# Autodesk Inventor assembly: 000.400 - Рычаг 2
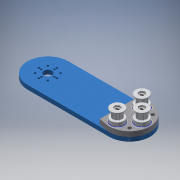
[picture p0: Inventor's stored thumbnail of the model, 180x180]
Saved by Autodesk Inventor 2019 (Build 230136000, 136)
## iProperties
Created: 2020-03-18
Part Number: 000.400 - Рычаг 2
Material: Типовые
Document SubType Name: Assembly
Designer: Петров Иван
Author: Петров Иван
## Documents named in this file (6)
- E:\IVAN\Ivan_desktop\GitHub\Manipulation_IRS\hardware\SCARA\000.400 - Рычаг 2.iam
- E:\IVAN\Ivan_desktop\GitHub\Manipulation_IRS\hardware\SCARA\000.401 - Опорная платформа.ipt
- E:\IVAN\Ivan_desktop\GitHub\Manipulation_IRS\hardware\SCARA\components\Подшипник 626Z.ipt
- E:\IVAN\Ivan_desktop\GitHub\Manipulation_IRS\hardware\SCARA\000.403 -  Прижим подшипников.ipt
- E:\IVAN\Ivan_desktop\GitHub\Manipulation_IRS\hardware\SCARA\components\Timing Pulley 18T.ipt
- C:\Users\Петров Иван\Documents\Inventor\Content Center Files\R2019\ru-RU\CNS 3129\CNS 3129 - M 4 x 0,7.ipt
## Components (11 placed, 5 different names)
1. 000.401 - Опорная платформа:1 — Совмещение:1, Совмещение:2, Совмещение:3, Совмещение:4, Совмещение:5, Совмещение:6, Совмещение:7
2. Подшипник 626Z:1 — Совмещение:1, Совмещение:6, Совмещение:8, Совмещение:14, Совмещение:15
3. Подшипник 626Z:2 — Совмещение:2, Совмещение:4, Совмещение:9, Совмещение:12, Совмещение:13
4. Подшипник 626Z:3 — Совмещение:3, Совмещение:5, Совмещение:10, Совмещение:11
5. 000.403 -  Прижим подшипников:1 — Совмещение:7, Совмещение:8, Совмещение:9
6. Timing Pulley 18T:1 — Совмещение:10, Совмещение:11, Направление навивки:2, Совмещение:18, Совмещение:19, Угол:3
7. Timing Pulley 18T:2 — Совмещение:14, Совмещение:15, Направление навивки:1, Совмещение:16, Угол:2, Совмещение:17
8. Timing Pulley 18T:3 — Совмещение:12, Совмещение:13, Направление навивки:1, Направление навивки:2, Вставка:1, Угол:1
9. CNS 3129 M 4:1 — Вставка:1, Угол:1
10. CNS 3129 M 4:2 — Совмещение:16, Угол:2, Совмещение:17
11. CNS 3129 M 4:3 — Совмещение:18, Совмещение:19, Угол:3
## Relationships (25: Mate 19, Angle 3, RelateRotation 2, Insert 1)
- Совмещение:1 [Mate]: 000.401 - Опорная платформа:1 ↔ Подшипник 626Z:1
- Совмещение:2 [Mate]: 000.401 - Опорная платформа:1 ↔ Подшипник 626Z:2
- Совмещение:3 [Mate]: 000.401 - Опорная платформа:1 ↔ Подшипник 626Z:3
- Совмещение:4 [Mate]: 000.401 - Опорная платформа:1 ↔ Подшипник 626Z:2
- Совмещение:5 [Mate]: 000.401 - Опорная платформа:1 ↔ Подшипник 626Z:3
- Совмещение:6 [Mate]: 000.401 - Опорная платформа:1 ↔ Подшипник 626Z:1
- Совмещение:7 [Mate]: 000.401 - Опорная платформа:1 ↔ 000.403 -  Прижим подшипников:1
- Совмещение:8 [Mate]: Подшипник 626Z:1 ↔ 000.403 -  Прижим подшипников:1
- Совмещение:9 [Mate]: Подшипник 626Z:2 ↔ 000.403 -  Прижим подшипников:1
- Совмещение:10 [Mate]: Подшипник 626Z:3 ↔ Timing Pulley 18T:1
- Совмещение:11 [Mate]: Подшипник 626Z:3 ↔ Timing Pulley 18T:1
- Совмещение:12 [Mate]: Подшипник 626Z:2 ↔ Timing Pulley 18T:3
- Совмещение:13 [Mate]: Подшипник 626Z:2 ↔ Timing Pulley 18T:3
- Совмещение:14 [Mate]: Подшипник 626Z:1 ↔ Timing Pulley 18T:2
- Совмещение:15 [Mate]: Подшипник 626Z:1 ↔ Timing Pulley 18T:2
- Направление навивки:1 [RelateRotation] (1 ul): Timing Pulley 18T:2 ↔ Timing Pulley 18T:3
- Направление навивки:2 [RelateRotation] (1 ul): Timing Pulley 18T:1 ↔ Timing Pulley 18T:3
- Вставка:1 [Insert]: Timing Pulley 18T:3 ↔ CNS 3129 M 4:1
- Угол:1 [Angle] (0 deg): Timing Pulley 18T:3 ↔ CNS 3129 M 4:1
- Совмещение:16 [Mate]: Timing Pulley 18T:2 ↔ CNS 3129 M 4:2
- Угол:2 [Angle] (0 deg): Timing Pulley 18T:2 ↔ CNS 3129 M 4:2
- Совмещение:17 [Mate]: Timing Pulley 18T:2 ↔ CNS 3129 M 4:2
- Совмещение:18 [Mate]: Timing Pulley 18T:1 ↔ CNS 3129 M 4:3
- Совмещение:19 [Mate]: Timing Pulley 18T:1 ↔ CNS 3129 M 4:3
- Угол:3 [Angle] (0 deg): Timing Pulley 18T:1 ↔ CNS 3129 M 4:3
